# Autodesk Inventor assembly: MIR_HbWrist
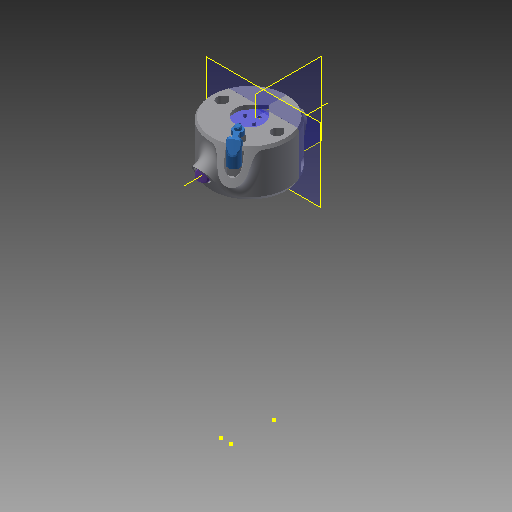
[picture p0: Inventor's stored thumbnail of the model, 512x512]
Saved by Autodesk Inventor 2018.1 (Build 221171000, 171)
## iProperties
Part Number: MIR_HbWrist
Material: 一般
Document SubType Name: Assembly
Designer: sktom
Author: sktom
## Documents named in this file (9)
- D:\CloudStrage\OneDrive\CAD\MAJ\hackberry\HACKberry-hardware\3D_69%inlength\Inventor\HbWristForChild\MIR_HbWrist.iam
- D:\CloudStrage\OneDrive\CAD\MAJ\hackberry\HACKberry-hardware\3D_69%inlength\Inventor\HbWristForChild\MIR_HBarmMountBase03ForChild.ipt
- D:\CloudStrage\OneDrive\CAD\MAJ\hackberry\HACKberry-hardware\3D_69%inlength\Inventor\HbWristForChild\MIR_HBlockPlateHolder02ForChild.ipt
- D:\CloudStrage\OneDrive\CAD\MAJ\hackberry\HACKberry-hardware\3D_69%inlength\Inventor\HbWristForChild\MIR_HBarmMount02ForChild.ipt
- D:\CloudStrage\OneDrive\CAD\MAJ\hackberry\HACKberry-hardware\3D_69%inlength\Inventor\HbWristForChild\MIR_HBpronationLockPin02ForChild.ipt
- D:\CloudStrage\OneDrive\CAD\MAJ\hackberry\HACKberry-hardware\3D_69%inlength\Inventor\HbWristForChild\MIR_HBejectorLever02ForChild.ipt
- D:\CloudStrage\OneDrive\CAD\MAJ\hackberry\HACKberry-hardware\3D_69%inlength\Inventor\HbWristForChild\MIR_HBabductionLever02forChild.ipt
- D:\CloudStrage\OneDrive\CAD\MAJ\hackberry\HACKberry-hardware\3D_69%inlength\Inventor\HbWristForChild\MIR_HBarmMountBaseCover03ForChild.ipt
- D:\CloudStrage\OneDrive\CAD\MAJ\hackberry\HACKberry-hardware\3D_69%inlength\Inventor\HbWristForChild\MIR_HbWristLockPlate01ForChild.ipt
## Components (8 placed, 8 different names)
1. MIR_HBarmMountBase03ForChild:1 — 挿入:1, フラッシュ:1, 挿入:3, 挿入:2, 円柱状:5, 円柱状:1
2. MIR_HBlockPlateHolder02ForChild:1 — 挿入:1, 挿入:5, 挿入:4
3. MIR_HBarmMount02ForChild:1 — メイト:1, 円柱状:7, 円柱状:2
4. MIR_HBpronationLockPin02ForChild:1 — 円柱状:5
5. MIR_HBejectorLever02ForChild:1 — 円柱状:7, 円柱状:2, 円柱状:6
6. MIR_HBabductionLever02forChild:1 — フラッシュ:1, 円柱状:6, 円柱状:1
7. MIR_HBarmMountBaseCover03ForChild:1 — メイト:1, 挿入:3, 挿入:2
8. MIR_HbWristLockPlate01ForChild:1 — 挿入:5, 挿入:4
## Relationships (12: Insert 5, CylindricalJoint 5, Flush 1, Mate 1)
- 挿入:1 [Insert]: MIR_HBarmMountBase03ForChild:1 ↔ MIR_HBlockPlateHolder02ForChild:1
- フラッシュ:1 [Flush]: MIR_HBarmMountBase03ForChild:1 ↔ MIR_HBabductionLever02forChild:1
- メイト:1 [Mate] (0.1 mm): MIR_HBarmMount02ForChild:1 ↔ MIR_HBarmMountBaseCover03ForChild:1
- 挿入:3 [Insert]: MIR_HBarmMountBase03ForChild:1 ↔ MIR_HBarmMountBaseCover03ForChild:1
- 挿入:2 [Insert]: MIR_HBarmMountBase03ForChild:1 ↔ MIR_HBarmMountBaseCover03ForChild:1
- 挿入:5 [Insert]: MIR_HBlockPlateHolder02ForChild:1 ↔ MIR_HbWristLockPlate01ForChild:1
- 挿入:4 [Insert]: MIR_HBlockPlateHolder02ForChild:1 ↔ MIR_HbWristLockPlate01ForChild:1
- 円柱状:5 [CylindricalJoint]: MIR_HBarmMountBase03ForChild:1 ↔ MIR_HBpronationLockPin02ForChild:1
- 円柱状:7 [CylindricalJoint]: MIR_HBarmMount02ForChild:1 ↔ MIR_HBejectorLever02ForChild:1
- 円柱状:2 [CylindricalJoint]: MIR_HBarmMount02ForChild:1 ↔ MIR_HBejectorLever02ForChild:1
- 円柱状:6 [CylindricalJoint]: MIR_HBejectorLever02ForChild:1 ↔ MIR_HBabductionLever02forChild:1
- 円柱状:1 [CylindricalJoint]: MIR_HBarmMountBase03ForChild:1 ↔ MIR_HBabductionLever02forChild:1
